# Autodesk Inventor assembly: Arm for Gen 2
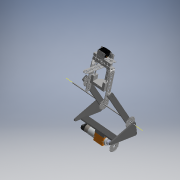
[picture p0: Inventor's stored thumbnail of the model, 180x180]
Saved by Autodesk Inventor 2019 (Build 230136000, 136)
## iProperties
Part Number: Arm for Gen 2
Document SubType Name: Assembly
Designer: Delta
Author: Delta
## Documents named in this file (10)
- C:\Robotics\CAD\2019-20_CAD\Collection\Arm for Gen 2.iam
- C:\Robotics\CAD\2019-20_CAD\Collection\12 Inch Hex Axle.ipt
- C:\Robotics\CAD\COTSParts\Sprockets - AndyMark\615106.ipt
- C:\Robotics\CAD\2019-20_CAD\Collection\bar arms.ipt
- C:\Robotics\CAD\2019-20_CAD\Collection\Spacer .25D .375H.ipt
- C:\Robotics\CAD\2019-20_CAD\Collection\Motor mount bar.ipt
- C:\Robotics\CAD\COTSParts\Motors\am-3643 NeveRest Sport, 104-1 with Motor.ipt
- C:\Robotics\CAD\2019-20_CAD\Collection\Motor spacer.ipt
- C:\Robotics\CAD\2019-20_CAD\Collection\The Claw.iam
- C:\Robotics\CAD\2019-20_CAD\Collection\Triangle axle slide connector.ipt
## Components (13 placed, 9 different names)
1. 12 Inch Hex Axle:1 — Mate:5, Mate:6, Mate:8, Mate:55, Mate:74, Flush:13, Mate:102, Mate:103
2. 615106:1 — Mate:5, Flush:12
3. bar arms:1 — Mate:6, Flush:5, Mate:90, Mate:94, Mate:95, Mate:105
4. bar arms:2 — Mate:8, Flush:5, Mate:54, Mate:93, Flush:13, angle of arms
5. Spacer .25D .375H:1 — Mate:54, Mate:55
6. Motor mount bar:1 — Flush:8, Mate:70, Mate:79, Mate:97, Mate:98, Mate:99, Mate:101, Mate:104
7. am-3643 NeveRest Sport, 104-1 with Motor:1 — Flush:6, Flush:7, Mate:72, Mate:73, Mate:82, Angle:1
8. Motor spacer:1 — Flush:6, Flush:7, Flush:8, Mate:70, Mate:73, Mate:79
9. 615106:3 — Mate:72, Mate:82, Flush:12
10. 615106:4 — Mate:74, Mate:90
11. The Claw:1 [sub-assembly] — Mate:93, Mate:94, Mate:95, Angle:1
12. Triangle axle slide connector:1 — Mate:101, Mate:102, Mate:104, Mate:105
13. Triangle axle slide connector:2 — Mate:97, Mate:98, Mate:99, Mate:103, angle of arms
## Relationships (31: Mate 23, Flush 6, Angle 2)
- Mate:5: 12 Inch Hex Axle:1 ↔ 615106:1
- Mate:6: 12 Inch Hex Axle:1 ↔ bar arms:1
- Mate:8: 12 Inch Hex Axle:1 ↔ bar arms:2
- Flush:5: bar arms:1 ↔ bar arms:2
- Mate:54: bar arms:2 ↔ Spacer .25D .375H:1
- Mate:55: 12 Inch Hex Axle:1 ↔ Spacer .25D .375H:1
- Flush:6: am-3643 NeveRest Sport, 104-1 with Motor:1 ↔ Motor spacer:1
- Flush:7: am-3643 NeveRest Sport, 104-1 with Motor:1 ↔ Motor spacer:1
- Flush:8: Motor mount bar:1 ↔ Motor spacer:1
- Mate:70: Motor mount bar:1 ↔ Motor spacer:1
- Mate:72: am-3643 NeveRest Sport, 104-1 with Motor:1 ↔ 615106:3
- Mate:73: am-3643 NeveRest Sport, 104-1 with Motor:1 ↔ Motor spacer:1
- Mate:74: 12 Inch Hex Axle:1 ↔ 615106:4
- Mate:79: Motor mount bar:1 ↔ Motor spacer:1
- Mate:82 (25.4 mm): am-3643 NeveRest Sport, 104-1 with Motor:1 ↔ 615106:3
- Mate:90 (9.6266 mm): bar arms:1 ↔ 615106:4
- Flush:12: 615106:1 ↔ 615106:3
- Mate:93: bar arms:2 ↔ The Claw:1
- Mate:94: bar arms:1 ↔ The Claw:1
- Mate:95: bar arms:1 ↔ The Claw:1
- Angle:1 (0.1 deg): am-3643 NeveRest Sport, 104-1 with Motor:1 ↔ The Claw:1
- Flush:13 (-44.45 mm): 12 Inch Hex Axle:1 ↔ bar arms:2
- Mate:97: Motor mount bar:1 ↔ Triangle axle slide connector:2
- Mate:98: Motor mount bar:1 ↔ Triangle axle slide connector:2
- Mate:99: Motor mount bar:1 ↔ Triangle axle slide connector:2
- Mate:101: Motor mount bar:1 ↔ Triangle axle slide connector:1
- Mate:102: 12 Inch Hex Axle:1 ↔ Triangle axle slide connector:1
- Mate:103: 12 Inch Hex Axle:1 ↔ Triangle axle slide connector:2
- Mate:104: Motor mount bar:1 ↔ Triangle axle slide connector:1
- Mate:105 (12.7 mm): bar arms:1 ↔ Triangle axle slide connector:1
- angle of arms (20 deg): bar arms:2 ↔ Triangle axle slide connector:2
